# Autodesk Inventor assembly: UBG-Rolle
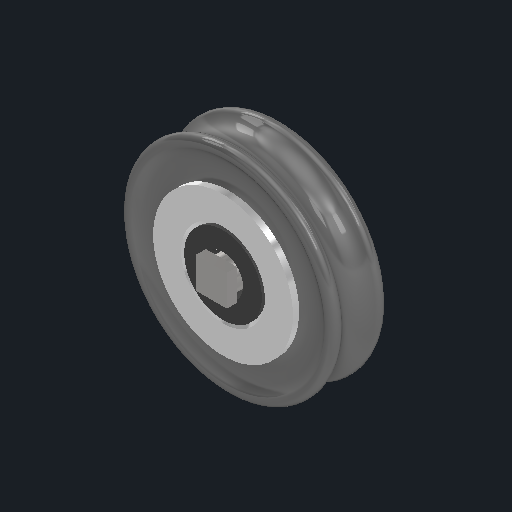
[picture p0: Inventor's stored thumbnail of the model, 512x512]
Saved by Autodesk Inventor 2026.1 (Build 301233000, 233)
## iProperties
Created: 2024-11-07
Part Number: UBG-Rolle
Document SubType Name: Assembly
Designer: Fabian
Author: Fabian
## Documents named in this file (5)
- C:\Users\JurijLenz\Nextcloud\Jurij treibt Dinge (keine Kamele)\RadLWL\Rolle\UBG-Rolle.iam
- C:\Users\JurijLenz\Nextcloud\Jurij treibt Dinge (keine Kamele)\RadLWL\Rolle\Gleitlager MSM-0205-02.ipt
- C:\Users\JurijLenz\Nextcloud\Jurij treibt Dinge (keine Kamele)\RadLWL\Rolle\Rolle.ipt
- C:\Users\JurijLenz\Nextcloud\Jurij treibt Dinge (keine Kamele)\RadLWL\Rolle\Welle Querrolle Quad.ipt
- C:\Users\JurijLenz\Nextcloud\Jurij treibt Dinge (keine Kamele)\RadLWL\Rolle\X-Ring 5.94x3.53.ipt
## Components (5 placed, 4 different names)
1. Rolle:1 — Fluchtend:1, Passend:1, Passend:2, Passend:3, Passend:4, Fluchtend:2, Fluchtend:3, Passend:5
2. X-Ring 5.94x3.53:1 — Passend:3
3. Gleitlager MSM-0205-02:1 — Passend:4, Fluchtend:2
4. Gleitlager MSM-0205-02:2 — Fluchtend:3, Passend:5, Passend:6
5. Welle Querrolle Quad:1 — Passend:6, Passend:7, Winkel:1
## Relationships (11: Mate 7, Flush 3, Angle 1)
- Fluchtend:1 [Flush] (-2 mm): Rolle:1
- Passend:1 [Mate]: Rolle:1
- Passend:2 [Mate]: Rolle:1
- Passend:3 [Mate]: Rolle:1 ↔ X-Ring 5.94x3.53:1
- Passend:4 [Mate]: Rolle:1 ↔ Gleitlager MSM-0205-02:1
- Fluchtend:2 [Flush]: Rolle:1 ↔ Gleitlager MSM-0205-02:1
- Fluchtend:3 [Flush]: Rolle:1 ↔ Gleitlager MSM-0205-02:2
- Passend:5 [Mate]: Rolle:1 ↔ Gleitlager MSM-0205-02:2
- Passend:6 [Mate]: Gleitlager MSM-0205-02:2 ↔ Welle Querrolle Quad:1
- Passend:7 [Mate]: Welle Querrolle Quad:1
- Winkel:1 [Angle] (0 deg): Welle Querrolle Quad:1
